# Autodesk Inventor assembly: ASY TZS 1650 filter-distribution-system 940
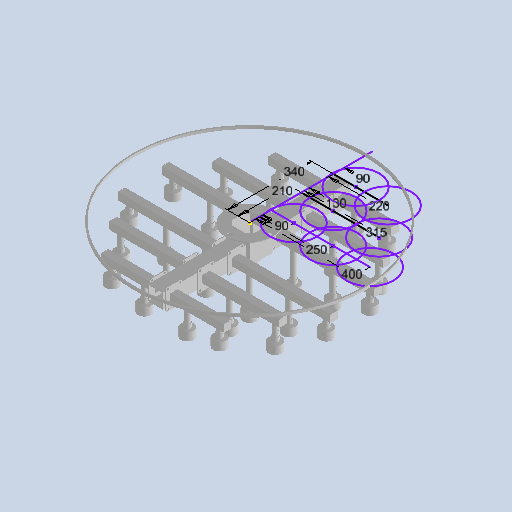
[picture p0: Inventor's stored thumbnail of the model, 512x512]
Saved by Autodesk Inventor 2025 (Build 290162010, 162A)
## iProperties
Created: 2025-06-24
Part Number: ASY TZS 1650 filter-distribution-system 940
Document SubType Name: Assembly
Designer: admin
Author: user
## Documents named in this file (9)
- C:\Users\pokla\Documents\Inventor\TZS-Tazovskiy\Filter D940\FDS 940\ASY TZS 1650 filter-distribution-system 940.iam
- C:\Users\pokla\Documents\Inventor\TZS-Tazovskiy\Filter D940\FDS 940\TZS 169859 DIM filter-distribution-system 940.ipt
- C:\Users\pokla\Documents\Inventor\TZS-Tazovskiy\Filter D940\FDS 940\TZS 1651 FDS MAIN  FLANGE.ipt
- C:\Users\pokla\Documents\Inventor\TZS-Tazovskiy\Filter D940\FDS 940\TZS 1652 FDS Central tube wall.ipt
- C:\Users\pokla\Documents\Inventor\TZS-Tazovskiy\Filter D940\FDS 940\TZS 1653 FDS 940 Diameter beam.ipt
- C:\Users\pokla\Documents\Inventor\TZS-Tazovskiy\Filter D940\FDS 940\ASY TZS FDS way1_940.iam
- C:\Users\pokla\Documents\Inventor\TZS-Tazovskiy\Filter D940\FDS 940\ASY TZS 1662 FDS way 2.iam
- C:\Users\pokla\Documents\Inventor\TZS-Tazovskiy\Filter D940\FDS 940\ASY TZS FDS way3_940.iam
- C:\Users\pokla\Documents\Inventor\TZS-Tazovskiy\Filter D940\FDS 940\TZS 1665 FDS 940 CUP 1.ipt
## Components (19 placed, 8 different names)
1. TZS 169859 DIM filter-distribution-system 940.ipt:1 — Mate:5, Mate:4
2. TZS 1651 FDS MAIN  FLANGE.ipt:1 — Flush:1, Flush:2, Mate:1
3. TZS 1652 FDS Central tube wall.ipt:1 — Flush:1, Flush:4, Flush:3, Mate:6, Rigid:1, Rigid:2
4. TZS 1652 FDS Central tube wall.ipt:2 — Flush:2, Mate:1, Rigid:1, Rigid:3
5. TZS 1653 FDS 940 Diameter beam.ipt:1 — Rigid:2, Rigid:4, Rigid:5, Rigid:9, Rigid:14, Rigid:15, Rigid:35
6. TZS 1653 FDS 940 Diameter beam.ipt:2 — Rigid:3, Rigid:11, Rigid:13, Rigid:12, Rigid:16, Rigid:17, Rigid:34
7. ASY TZS FDS way1_940.iam:1 [sub-assembly] — Rigid:4
8. ASY TZS 1662 FDS way 2.iam:1 [sub-assembly] — Rigid:5
9. ASY TZS FDS way3_940.iam:1 [sub-assembly] — Rigid:35
10. ASY TZS FDS way1_940.iam:2 [sub-assembly] — Rigid:9
11. ASY TZS FDS way1_940.iam:3 [sub-assembly] — Rigid:11
12. ASY TZS 1662 FDS way 2.iam:2 [sub-assembly] — Rigid:14
13. ASY TZS 1662 FDS way 2.iam:3 [sub-assembly] — Rigid:13
14. ASY TZS 1662 FDS way 2.iam:4 [sub-assembly] — Rigid:12
15. ASY TZS FDS way3_940.iam:2 [sub-assembly] — Rigid:15
16. ASY TZS FDS way3_940.iam:3 [sub-assembly] — Rigid:16
17. ASY TZS FDS way3_940.iam:4 [sub-assembly] — Rigid:17
18. TZS 1665 FDS 940 CUP 1.ipt:1 — Flush:4, Flush:3, Mate:6
19. ASY TZS FDS way1_940.iam:4 [sub-assembly] — Rigid:34
## Relationships (23: WeldJoint 15, Mate 4, Flush 4)
- Mate:5: TZS 169859 DIM filter-distribution-system 940.ipt:1
- Mate:4: TZS 169859 DIM filter-distribution-system 940.ipt:1
- Flush:1: TZS 1651 FDS MAIN  FLANGE.ipt:1 ↔ TZS 1652 FDS Central tube wall.ipt:1
- Flush:2: TZS 1651 FDS MAIN  FLANGE.ipt:1 ↔ TZS 1652 FDS Central tube wall.ipt:2
- Mate:1: TZS 1651 FDS MAIN  FLANGE.ipt:1 ↔ TZS 1652 FDS Central tube wall.ipt:2
- Flush:4: TZS 1652 FDS Central tube wall.ipt:1 ↔ TZS 1665 FDS 940 CUP 1.ipt:1
- Flush:3: TZS 1652 FDS Central tube wall.ipt:1 ↔ TZS 1665 FDS 940 CUP 1.ipt:1
- Mate:6: TZS 1652 FDS Central tube wall.ipt:1 ↔ TZS 1665 FDS 940 CUP 1.ipt:1
- Rigid:1 [WeldJoint]: TZS 1652 FDS Central tube wall.ipt:1 ↔ TZS 1652 FDS Central tube wall.ipt:2
- Rigid:2 [WeldJoint]: TZS 1652 FDS Central tube wall.ipt:1 ↔ TZS 1653 FDS 940 Diameter beam.ipt:1
- Rigid:3 [WeldJoint]: TZS 1652 FDS Central tube wall.ipt:2 ↔ TZS 1653 FDS 940 Diameter beam.ipt:2
- Rigid:4 [WeldJoint] (-2 mm): TZS 1653 FDS 940 Diameter beam.ipt:1 ↔ ASY TZS FDS way1_940.iam:1
- Rigid:5 [WeldJoint] (-2 mm): TZS 1653 FDS 940 Diameter beam.ipt:1 ↔ ASY TZS 1662 FDS way 2.iam:1
- Rigid:9 [WeldJoint]: TZS 1653 FDS 940 Diameter beam.ipt:1 ↔ ASY TZS FDS way1_940.iam:2
- Rigid:11 [WeldJoint]: TZS 1653 FDS 940 Diameter beam.ipt:2 ↔ ASY TZS FDS way1_940.iam:3
- Rigid:14 [WeldJoint]: TZS 1653 FDS 940 Diameter beam.ipt:1 ↔ ASY TZS 1662 FDS way 2.iam:2
- Rigid:13 [WeldJoint]: TZS 1653 FDS 940 Diameter beam.ipt:2 ↔ ASY TZS 1662 FDS way 2.iam:3
- Rigid:12 [WeldJoint]: TZS 1653 FDS 940 Diameter beam.ipt:2 ↔ ASY TZS 1662 FDS way 2.iam:4
- Rigid:15 [WeldJoint]: TZS 1653 FDS 940 Diameter beam.ipt:1 ↔ ASY TZS FDS way3_940.iam:2
- Rigid:16 [WeldJoint]: TZS 1653 FDS 940 Diameter beam.ipt:2 ↔ ASY TZS FDS way3_940.iam:3
- Rigid:17 [WeldJoint]: TZS 1653 FDS 940 Diameter beam.ipt:2 ↔ ASY TZS FDS way3_940.iam:4
- Rigid:34 [WeldJoint]: TZS 1653 FDS 940 Diameter beam.ipt:2 ↔ ASY TZS FDS way1_940.iam:4
- Rigid:35 [WeldJoint]: TZS 1653 FDS 940 Diameter beam.ipt:1 ↔ ASY TZS FDS way3_940.iam:1
